# Autodesk Inventor assembly: plate
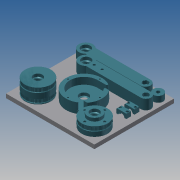
[picture p0: Inventor's stored thumbnail of the model, 180x180]
Saved by Autodesk Inventor 2013 (Build 170138000, 138)
## iProperties
Created: 2017-04-01
Part Number: plate
Document SubType Name: Assembly
Designer: employee
Author: employee
## Documents named in this file (9)
- C:\Users\employee\Desktop\SCARA\plate.iam
- C:\Users\employee\Desktop\SCARA\build plate.ipt
- C:\Users\employee\Desktop\SCARA\z idler pulley 2.ipt
- C:\Users\employee\Desktop\SCARA\proximal thin arm.ipt
- C:\Users\employee\Desktop\SCARA\driven arm.ipt
- C:\Users\employee\Desktop\SCARA\distal drive pulley.ipt
- C:\Users\employee\Desktop\SCARA\central pivot spacer.ipt
- C:\Users\employee\Desktop\SCARA\e3d mount.ipt
- C:\Users\employee\Desktop\SCARA\offset shield.ipt
## Components (9 placed, 8 different names)
1. build plate:1 — Mate:1, Mate:2, Mate:3, Mate:4, Mate:5, Mate:6, Mate:7, Mate:8
2. z idler pulley 2:1 — Mate:1
3. proximal thin arm:1 — Mate:2
4. driven arm:1 — Mate:3
5. distal drive pulley:1 — Mate:4
6. central pivot spacer:1 — Mate:5
7. e3d mount:1 — Mate:7
8. e3d mount:2 — Mate:6
9. offset shield:1 — Mate:8
## Relationships (8: Mate 8)
- Mate:1: build plate:1 ↔ z idler pulley 2:1
- Mate:2: build plate:1 ↔ proximal thin arm:1
- Mate:3: build plate:1 ↔ driven arm:1
- Mate:4: build plate:1 ↔ distal drive pulley:1
- Mate:5: build plate:1 ↔ central pivot spacer:1
- Mate:6: build plate:1 ↔ e3d mount:2
- Mate:7: build plate:1 ↔ e3d mount:1
- Mate:8: build plate:1 ↔ offset shield:1
